# Autodesk Inventor assembly: Arm 1.1
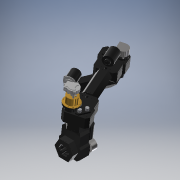
[picture p0: Inventor's stored thumbnail of the model, 180x180]
Saved by Autodesk Inventor 2017 (Build 210142000, 142)
## iProperties
Created: 2019-09-19
Part Number: Arm 1.1
Document SubType Name: Assembly
Designer: Dell
Author: Dell
## Documents named in this file (5)
- C:\Users\Dell\Documents\GitHub\tr2\Arm 1.1\Arm 1.1.iam
- C:\Users\Dell\Documents\GitHub\tr2\Arm 1.1\A01.ipt
- C:\Users\Dell\Documents\GitHub\tr2\Arm 1.1\A02.ipt
- C:\Users\Dell\Documents\GitHub\tr2\Actuator 2.0\XT-40.iam
- C:\Users\Dell\Documents\GitHub\tr2\Actuator 2.0\XT-6.iam
## Components (5 placed, 4 different names)
1. XT-40:1 [sub-assembly] — Mate:37, Mate:38, Mate:39, Mate:40, Mate:41
2. XT-40:2 [sub-assembly] — Mate:48, Mate:49, Mate:50, Mate:51
3. XT-6:1 [sub-assembly] — Mate:44, Mate:45, Mate:46, Mate:47, Mate:49, Mate:51
4. A01:1 — Mate:37, Mate:38, Mate:39, Mate:44, Mate:45, Mate:46, Mate:47
5. A02:1 — Mate:40, Mate:41
## Relationships (13: Mate 13)
- Mate:37: XT-40:1 ↔ A01:1
- Mate:38: XT-40:1 ↔ A01:1
- Mate:39: XT-40:1 ↔ A01:1
- Mate:40: XT-40:1 ↔ A02:1
- Mate:41: XT-40:1 ↔ A02:1
- Mate:44: XT-6:1 ↔ A01:1
- Mate:45: XT-6:1 ↔ A01:1
- Mate:46: XT-6:1 ↔ A01:1
- Mate:47: XT-6:1 ↔ A01:1
- Mate:48: XT-40:2
- Mate:49: XT-40:2 ↔ XT-6:1
- Mate:50: XT-40:2
- Mate:51: XT-40:2 ↔ XT-6:1
